# Autodesk Inventor assembly: motor
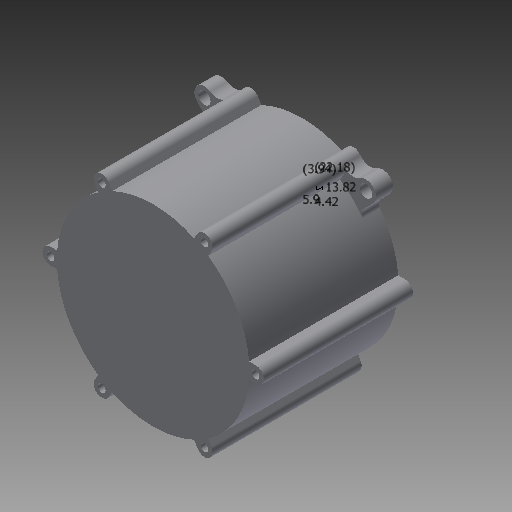
[picture p0: Inventor's stored thumbnail of the model, 512x512]
Saved by Autodesk Inventor 2019.3 (Build 233278000, 278)
## iProperties
Created: 2017-11-28
Part Number: motor
Document SubType Name: Assembly
Designer: eroldan
Author: eroldan
## Documents named in this file (3)
- C:\Users\eroldan\Desktop\3dprojects\OpenEmoto\OtherParts\BigBlock.iam
- C:\Users\eroldan\Desktop\3dprojects\OpenEmoto\OtherParts\BigBlock.ipt
- C:\Users\eroldan\Desktop\3dprojects\OpenEmoto\OtherParts\DriveSprocket12T.ipt
## Components (2 placed, 2 different names)
1. BigBlock:1 — Mate:1, Flush:1
2. DriveSprocket12T:1 — Mate:1, Flush:1
## Relationships (2: Mate 1, Flush 1)
- Mate:1: BigBlock:1 ↔ DriveSprocket12T:1
- Flush:1 (27 mm): BigBlock:1 ↔ DriveSprocket12T:1
